# Autodesk Inventor assembly: Биореактор_сборка
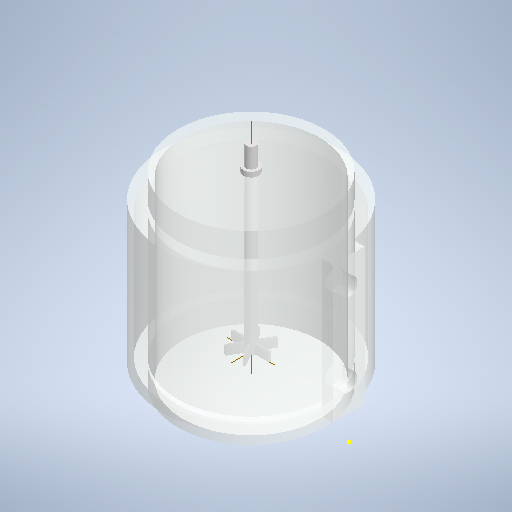
[picture p0: Inventor's stored thumbnail of the model, 512x512]
Saved by Autodesk Inventor 2025 (Build 290162000, 162)
## iProperties
Created: 2026-05-30
Part Number: Биореактор_сборка
Document SubType Name: Assembly
Designer: User
Author: User
## Documents named in this file (3)
- C:\Users\User\Downloads\Биореактор_сборка.iam
- C:\Users\User\Downloads\Корпус биореактора с рубашкой.ipt
- C:\Users\User\Downloads\Мешалка.ipt
## Components (2 placed, 2 different names)
1. Корпус биореактора с рубашкой:1 — Вставка:1
2. Мешалка:1 — Вставка:1, Совмещение:1
## Relationships (2: Insert 1, Mate 1)
- Вставка:1 [Insert]: Корпус биореактора с рубашкой:1 ↔ Мешалка:1
- Совмещение:1 [Mate]: Мешалка:1
